# Autodesk Inventor assembly: PieDeBomba
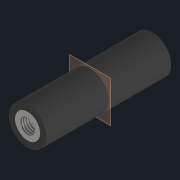
[picture p0: Inventor's stored thumbnail of the model, 180x180]
Saved by Autodesk Inventor 2021 (Build 250183000, 183)
## iProperties
Created: 2021-06-01
Part Number: PieDeBomba
Document SubType Name: Assembly
Designer: GABRIEL LOL
Author: GABRIEL LOL
## Documents named in this file (3)
- C:\Users\GABRIEL LOL\Desktop\planos pai\PieDeBomba.iam
- C:\Users\GABRIEL LOL\Desktop\planos pai\PataPolimero.ipt
- C:\Users\GABRIEL LOL\Desktop\planos pai\RoscaPataPolimero.ipt
## Components (3 placed, 2 different names)
1. PataPolimero:1 — Mate:1, Flush:1, Mate:2, Flush:2
2. RoscaPataPolimero:1 — Mate:1, Flush:1
3. RoscaPataPolimero:2 — Mate:2, Flush:2
## Relationships (4: Mate 2, Flush 2)
- Mate:1: PataPolimero:1 ↔ RoscaPataPolimero:1
- Flush:1: PataPolimero:1 ↔ RoscaPataPolimero:1
- Mate:2: PataPolimero:1 ↔ RoscaPataPolimero:2
- Flush:2: PataPolimero:1 ↔ RoscaPataPolimero:2
